# Autodesk Inventor assembly: 조립도
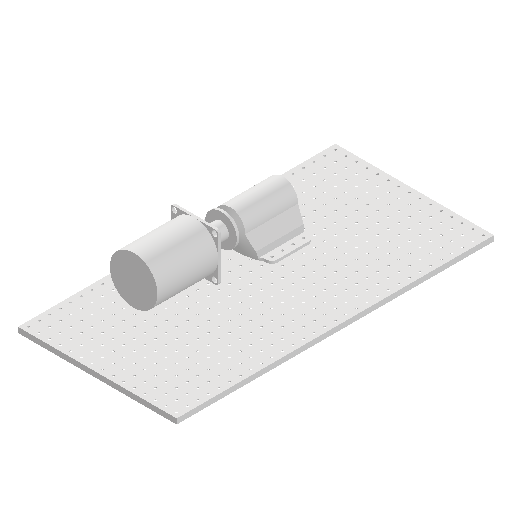
[picture p0: Inventor's stored thumbnail of the model, 512x512]
Saved by Autodesk Inventor 2027 (Build 310192000, 192)
## iProperties
Created: 2026-09-29
Part Number: 조립도
Document SubType Name: Assembly
Designer: User
Author: User
## Documents named in this file (8)
- C:\Users\User\Desktop\4_권도영\졸업작품\INVENTOR\리프트_회전부\조립도.iam
- C:\Users\User\Desktop\4_권도영\졸업작품\INVENTOR\리프트_회전부\판넬.ipt
- C:\Users\User\Desktop\4_권도영\졸업작품\INVENTOR\리프트_회전부\바깥쪽_베어링 고정부_split1.ipt
- C:\Users\User\Desktop\4_권도영\졸업작품\INVENTOR\리프트_회전부\안쪽_베어링 고정부.ipt
- C:\Users\User\Desktop\4_권도영\졸업작품\INVENTOR\리프트_회전부\베어링.ipt
- C:\Users\User\Desktop\4_권도영\졸업작품\INVENTOR\리프트_회전부\바깥쪽_베어링 고정부_split2.ipt
- C:\Users\User\Desktop\4_권도영\졸업작품\INVENTOR\리프트_회전부\도르래.ipt
- C:\Users\User\Desktop\4_권도영\졸업작품\INVENTOR\리프트_회전부\모터.ipt
## Components (7 placed, 7 different names)
1. 판넬:1 — 삽입:1, 삽입:2, 메이트:2
2. 바깥쪽_베어링 고정부_split1:1 — 삽입:1, 삽입:2, 메이트:1, 메이트:3, 플러쉬:1
3. 안쪽_베어링 고정부:1 — 삽입:3, 삽입:5
4. 베어링:1 — 삽입:3, 메이트:1
5. 바깥쪽_베어링 고정부_split2:1 — 메이트:2, 메이트:3, 플러쉬:1
6. 도르래:1 — 삽입:4, 메이트:4, 플러쉬:2, 삽입:5
7. 모터:1 — 삽입:4, 메이트:4, 플러쉬:2
## Relationships (11: Insert 5, Mate 4, Flush 2)
- 삽입:1 [Insert]: 판넬:1 ↔ 바깥쪽_베어링 고정부_split1:1
- 삽입:2 [Insert]: 판넬:1 ↔ 바깥쪽_베어링 고정부_split1:1
- 삽입:3 [Insert]: 안쪽_베어링 고정부:1 ↔ 베어링:1
- 메이트:1 [Mate]: 바깥쪽_베어링 고정부_split1:1 ↔ 베어링:1
- 메이트:2 [Mate]: 판넬:1 ↔ 바깥쪽_베어링 고정부_split2:1
- 메이트:3 [Mate]: 바깥쪽_베어링 고정부_split1:1 ↔ 바깥쪽_베어링 고정부_split2:1
- 플러쉬:1 [Flush]: 바깥쪽_베어링 고정부_split1:1 ↔ 바깥쪽_베어링 고정부_split2:1
- 삽입:4 [Insert]: 도르래:1 ↔ 모터:1
- 메이트:4 [Mate]: 도르래:1 ↔ 모터:1
- 플러쉬:2 [Flush]: 도르래:1 ↔ 모터:1
- 삽입:5 [Insert]: 안쪽_베어링 고정부:1 ↔ 도르래:1
